# Autodesk Inventor assembly: Raspberry Pi
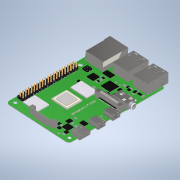
[picture p0: Inventor's stored thumbnail of the model, 180x180]
Saved by Autodesk Inventor 2020 (Build 240168000, 168)
## iProperties
Created: 2022-11-24
Part Number: Raspberry Pi
Document SubType Name: Assembly
Designer: DELL
Author: DELL
## Documents named in this file (7)
- C:\Users\DELL\OneDrive\Documents\Inventor\Raspberry Pi_Azzikri SSP_TFB\Pi.iam
- C:\Users\DELL\OneDrive\Documents\Inventor\Raspberry Pi_Azzikri SSP_TFB\Part2.ipt
- C:\Users\DELL\OneDrive\Documents\Inventor\Raspberry Pi_Azzikri SSP_TFB\Port 1.ipt
- C:\Users\DELL\OneDrive\Documents\Inventor\Raspberry Pi_Azzikri SSP_TFB\Port 2.ipt
- C:\Users\DELL\OneDrive\Documents\Inventor\Raspberry Pi_Azzikri SSP_TFB\Port 3.ipt
- C:\Users\DELL\OneDrive\Documents\Inventor\Raspberry Pi_Azzikri SSP_TFB\Port 4.ipt
- C:\Users\DELL\OneDrive\Documents\Inventor\Raspberry Pi_Azzikri SSP_TFB\Port 5.ipt
## Components (8 placed, 6 different names)
1. Part2:1 — Mate:2, Mate:3, Mate:4, Mate:5, Mate:6, Mate:7, Flush:1, Mate:8, Mate:9, Flush:2, Flush:3, Mate:10, Mate:11, Flush:4, Mate:12, Mate:13, Mate:14, Mate:15, Flush:5, Mate:16, Mate:17, Mate:18, Flush:6, Mate:19, Flush:7, Flush:8, Mate:20
2. Port 1:1 — Mate:6, Mate:7, Flush:1
3. Port 2:1 — Mate:4, Mate:5
4. Port 3:1 — Mate:17, Mate:18, Flush:6
5. Port 4:1 — Mate:12, Mate:13, Mate:14, Mate:15, Flush:5
6. Port 5:1 — Mate:8, Mate:9, Flush:2, Flush:3, Mate:10, Mate:11, Flush:4, Mate:16, Flush:8, Mate:20
7. Port 2:2 — Mate:2, Mate:3
8. Port 3:2 — Mate:19, Flush:7
## Relationships (27: Mate 19, Flush 8)
- Mate:2: Part2:1 ↔ Port 2:2
- Mate:3: Part2:1 ↔ Port 2:2
- Mate:4: Part2:1 ↔ Port 2:1
- Mate:5: Part2:1 ↔ Port 2:1
- Mate:6: Part2:1 ↔ Port 1:1
- Mate:7: Part2:1 ↔ Port 1:1
- Flush:1: Part2:1 ↔ Port 1:1
- Mate:8: Part2:1 ↔ Port 5:1
- Mate:9: Part2:1 ↔ Port 5:1
- Flush:2: Part2:1 ↔ Port 5:1
- Flush:3: Part2:1 ↔ Port 5:1
- Mate:10: Part2:1 ↔ Port 5:1
- Mate:11 (25.4 mm): Part2:1 ↔ Port 5:1
- Flush:4: Part2:1 ↔ Port 5:1
- Mate:12: Part2:1 ↔ Port 4:1
- Mate:13: Part2:1 ↔ Port 4:1
- Mate:14: Part2:1 ↔ Port 4:1
- Mate:15: Part2:1 ↔ Port 4:1
- Flush:5: Part2:1 ↔ Port 4:1
- Mate:16: Part2:1 ↔ Port 5:1
- Mate:17: Part2:1 ↔ Port 3:1
- Mate:18: Part2:1 ↔ Port 3:1
- Flush:6: Part2:1 ↔ Port 3:1
- Mate:19: Part2:1 ↔ Port 3:2
- Flush:7: Part2:1 ↔ Port 3:2
- Flush:8: Part2:1 ↔ Port 5:1
- Mate:20: Part2:1 ↔ Port 5:1
